# Autodesk Inventor assembly: ASY GBK 2130 short wall shield 3
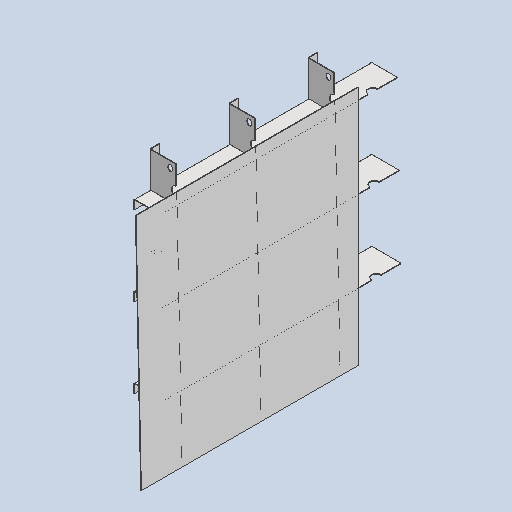
[picture p0: Inventor's stored thumbnail of the model, 512x512]
Saved by Autodesk Inventor 2026.3 (Build 303398000, 398)
## iProperties
Created: 2026-05-07
Part Number: ASY GBK 2130 short wall shield 3
Document SubType Name: Assembly
Designer: pokla
Stock Number: 2130
Mass: 136093 g
Surface Area: 87957.2 cm^2
Volume: 17336.7 cm^3
Density: 7.85 g/cm^3
Author: admin
Comments: поменял
## Documents named in this file (6)
- C:\Users\admin\Documents\Inventor\GBK-Gubkinskiy\ASY GBK 2130 short wall shield 3.iam
- C:\Users\admin\Documents\Inventor\GBK-Gubkinskiy\GBK 0101 main rib.ipt
- C:\Users\admin\Documents\Inventor\GBK-Gubkinskiy\GBK 0102 stringer 1.ipt
- C:\Users\admin\Documents\Inventor\GBK-Gubkinskiy\GBK 0103 stringer 2.ipt
- C:\Users\admin\Documents\Inventor\GBK-Gubkinskiy\GBK 0104 stringer 3.ipt
- C:\Users\admin\Documents\Inventor\GBK-Gubkinskiy\GBK 2133 shield 3.ipt
## Components (7 placed, 5 different names)
1. GBK 0101 main rib:1 — Mate:3, Mate:5, Rigid:1, Rigid:2, Rigid:3, Mate:5
2. GBK 0102 stringer 1:1 — Rigid:1, Rigid:4, Rigid:5
3. GBK 0103 stringer 2:1 — Rigid:2, Flush:2
4. GBK 0104 stringer 3:1 — Rigid:3
5. GBK 0101 main rib:2 — Rigid:4
6. GBK 0101 main rib:3 — Rigid:5
7. GBK 2133 shield 3:1 — Flush:1, Mate:5, Mate:6, Flush:2
## Relationships (11: WeldJoint 5, Mate 4, Flush 2)
- Mate:3: GBK 0101 main rib:1
- Mate:5: GBK 0101 main rib:1
- Rigid:1 [WeldJoint] (4 mm): GBK 0101 main rib:1 ↔ GBK 0102 stringer 1:1
- Rigid:2 [WeldJoint] (4 mm): GBK 0101 main rib:1 ↔ GBK 0103 stringer 2:1
- Rigid:3 [WeldJoint] (4 mm): GBK 0101 main rib:1 ↔ GBK 0104 stringer 3:1
- Rigid:4 [WeldJoint] (4 mm): GBK 0102 stringer 1:1 ↔ GBK 0101 main rib:2
- Rigid:5 [WeldJoint] (4 mm): GBK 0102 stringer 1:1 ↔ GBK 0101 main rib:3
- Flush:1: GBK 2133 shield 3:1
- Mate:5: GBK 0101 main rib:1 ↔ GBK 2133 shield 3:1
- Mate:6: GBK 2133 shield 3:1
- Flush:2 (155 mm): GBK 0103 stringer 2:1 ↔ GBK 2133 shield 3:1
